# Autodesk Inventor assembly: MG_996R
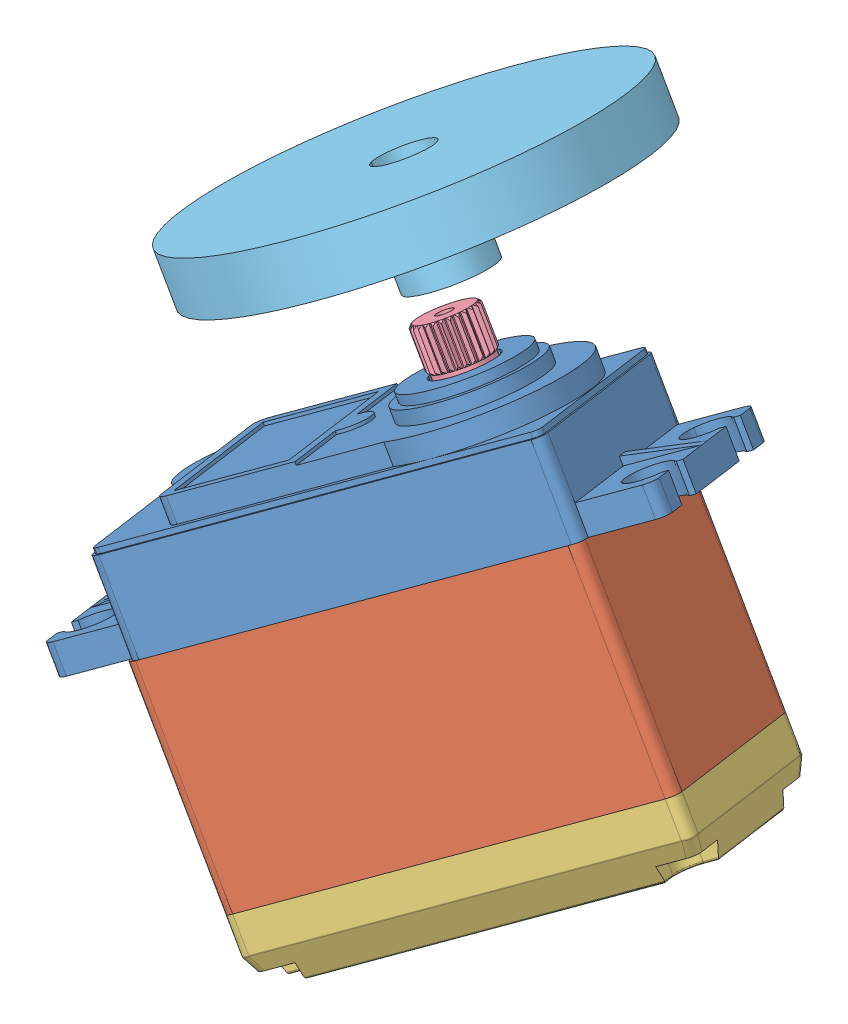
[picture p0: shaded view drawn from the shape stored in the file]
Saved by Autodesk Inventor 2025.2 (Build 292293000, 293)
## iProperties
Created: 2016-09-26
Part Number: MG_996R
Document SubType Name: Assembly
Designer: Julian
Author: Julian
## Documents named in this file (5)
- D:\Semester 2\Basics of Mechatronics\BO\MG_996R.iam
- D:\Semester 2\Basics of Mechatronics\BO\Base.ipt
- D:\Semester 2\Basics of Mechatronics\BO\Medio.ipt
- D:\Semester 2\Basics of Mechatronics\BO\Top.ipt
- D:\Semester 2\Basics of Mechatronics\BO\Eje.ipt
## Components (4 placed, 4 different names)
1. Top:1 — Rígido:2, De rotación:1
2. Medio:1 — Rígido:1, Rígido:2
3. Base:1 — Rígido:1
4. Eje:1 — De rotación:1
## Relationships (3: WeldJoint 2, RevoluteJoint 1)
- Rígido:1 [WeldJoint]: Medio:1 ↔ Base:1
- Rígido:2 [WeldJoint]: Top:1 ↔ Medio:1
- De rotación:1 [RevoluteJoint]: Top:1 ↔ Eje:1
